# Autodesk Inventor assembly: Leg3DOF
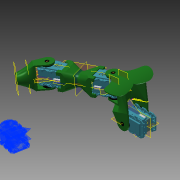
[picture p0: Inventor's stored thumbnail of the model, 180x180]
Saved by Autodesk Inventor 2015 (Build 190159000, 159)
## iProperties
Created: 2015-03-02
Part Number: Leg3DOF
Document SubType Name: Assembly
Designer: Henke
Author: Henke
## Documents named in this file (5)
- D:\Study_and_Projects\KTH\KEX i robotik\CAD\Leg3DOF.iam
- D:\Study_and_Projects\KTH\KEX i robotik\CAD\Servo with wheel.iam
- D:\Study_and_Projects\KTH\KEX i robotik\CAD\StraightConnector.ipt
- D:\Study_and_Projects\KTH\KEX i robotik\CAD\FootConnector.ipt
- D:\Study_and_Projects\KTH\KEX i robotik\CAD\HipConnector.ipt
## Components (6 placed, 4 different names)
1. Servo with wheel:1 [sub-assembly] — Rotational:1
2. Servo with wheel:2 [sub-assembly] — Rotational:2, Mate:7, Mate:9, Mate:11
3. Servo with wheel:3 [sub-assembly] — Mate:5, Mate:6, Mate:8, Mate:10, Mate:12
4. StraightConnector:1 — Mate:7, Mate:8, Mate:9, Mate:10, Mate:11, Mate:12
5. FootConnector:1 — Mate:5, Mate:6
6. HipConnector:1 — Rotational:1, Rotational:2
## Relationships (10: Mate 8, RevoluteJoint 2)
- Mate:5: Servo with wheel:3 ↔ FootConnector:1
- Mate:6: Servo with wheel:3 ↔ FootConnector:1
- Rotational:1 [RevoluteJoint]: Servo with wheel:1 ↔ HipConnector:1
- Rotational:2 [RevoluteJoint]: Servo with wheel:2 ↔ HipConnector:1
- Mate:7: Servo with wheel:2 ↔ StraightConnector:1
- Mate:8: Servo with wheel:3 ↔ StraightConnector:1
- Mate:9: Servo with wheel:2 ↔ StraightConnector:1
- Mate:10: Servo with wheel:3 ↔ StraightConnector:1
- Mate:11: Servo with wheel:2 ↔ StraightConnector:1
- Mate:12: Servo with wheel:3 ↔ StraightConnector:1
